# Autodesk Inventor assembly: Ankle_side_pitch
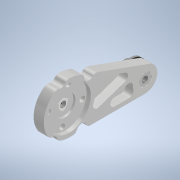
[picture p0: Inventor's stored thumbnail of the model, 180x180]
Saved by Autodesk Inventor 2020.4 (Build 244396000, 396)
## iProperties
Created: 2021-10-01
Part Number: Ankle_side_pitch
Document SubType Name: Assembly
Designer: Masato
Author: Masato
## Documents named in this file (7)
- C:\Users\Masato\Documents\Inventor\CIT Brains_Inventor\OpenPlatform_ver3_0（ワッシャ変更）\LowerBody\Ankle\Ankle_side_pitch.iam
- C:\Users\Masato\Documents\Inventor\CIT Brains_Inventor\OpenPlatform_ver3_0（ワッシャ変更）\LowerBody\Ankle\Ankle_side_pitch_frame.ipt
- C:\Users\Masato\Documents\Inventor\CIT Brains_Inventor\OpenPlatform_ver3_0（ワッシャ変更）\Ready_Made\UUW-0312-10BH.ipt
- C:\Users\Masato\Documents\Inventor\CIT Brains_Inventor\OpenPlatform_ver3_0（ワッシャ変更）\Ready_Made\S3-07-3W.ipt
- C:\Users\Masato\Documents\Inventor\CIT Brains_Inventor\OpenPlatform_ver3_0（ワッシャ変更）\Ready_Made\SF319.ipt
- C:\Users\Masato\Documents\Inventor\CIT Brains_Inventor\OpenPlatform_ver3_0（ワッシャ変更）\Ready_Made\CU-304.5H.ipt
- C:\Users\Masato\Documents\Inventor\CIT Brains_Inventor\OpenPlatform_ver3_0（ワッシャ変更）\Ready_Made\80F-0603.ipt
## Components (9 placed, 6 different names)
1. Ankle_side_pitch_frame:1 — 挿入:1, 角度:1, 挿入:2, 挿入:3, 挿入:4, フラッシュ:2, メイト:1
2. UUW-0312-10BH:1 — 挿入:3, 挿入:5, 挿入:8
3. UUW-0312-10BH:2 — 挿入:4, 挿入:6, 挿入:7
4. S3-07-3W:1 — 角度:1, 挿入:2
5. SF319:1 — 挿入:1, メイト:2
6. CU-304.5H:1 — 挿入:5
7. CU-304.5H:2 — 挿入:6
8. 80F-0603:1 — 挿入:7
9. 80F-0603:2 — 挿入:8
## Relationships (12: Insert 8, Mate 2, Angle 1, Flush 1)
- 挿入:1 [Insert]: Ankle_side_pitch_frame:1 ↔ SF319:1
- 角度:1 [Angle] (0 deg): Ankle_side_pitch_frame:1 ↔ S3-07-3W:1
- 挿入:2 [Insert]: Ankle_side_pitch_frame:1 ↔ S3-07-3W:1
- 挿入:3 [Insert]: Ankle_side_pitch_frame:1 ↔ UUW-0312-10BH:1
- 挿入:4 [Insert]: Ankle_side_pitch_frame:1 ↔ UUW-0312-10BH:2
- 挿入:5 [Insert]: UUW-0312-10BH:1 ↔ CU-304.5H:1
- 挿入:6 [Insert]: UUW-0312-10BH:2 ↔ CU-304.5H:2
- フラッシュ:2 [Flush]: Ankle_side_pitch_frame:1
- メイト:1 [Mate]: Ankle_side_pitch_frame:1
- メイト:2 [Mate]: SF319:1
- 挿入:7 [Insert]: UUW-0312-10BH:2 ↔ 80F-0603:1
- 挿入:8 [Insert]: UUW-0312-10BH:1 ↔ 80F-0603:2
